# Autodesk Inventor assembly: WinchNM
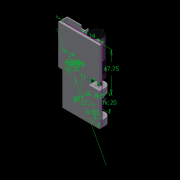
[picture p0: Inventor's stored thumbnail of the model, 180x180]
Saved by Autodesk Inventor 2019 (Build 230136000, 136)
## iProperties
Created: 2019-04-19
Part Number: WinchNM
Document SubType Name: Assembly
Designer: skylercleland
Author: skylercleland
## Documents named in this file (10)
- I:\FILES\School\12\DE\Projects\FinalProject\CAD\ShoeWinch\WinchNM.iam
- I:\FILES\School\12\DE\Projects\FinalProject\CAD\ShoeWinch\Bearing(8mm).ipt
- I:\FILES\School\12\DE\Projects\FinalProject\CAD\ShoeWinch\Bearing(608).ipt
- I:\FILES\School\12\DE\Projects\FinalProject\CAD\ShoeWinch\Part3.ipt
- I:\FILES\School\12\DE\Projects\FinalProject\CAD\ShoeWinch\Winch\Design Accelerator\Shaft2.iam
- I:\FILES\School\12\DE\Projects\FinalProject\CAD\ShoeWinch\Winch\Design Accelerator\Worm Gears2.iam
- I:\FILES\School\12\DE\Projects\FinalProject\CAD\ShoeWinch\Winch\Design Accelerator\Spur Gears2.iam
- I:\FILES\School\12\DE\Projects\FinalProject\CAD\ShoeWinch\LimitSwitch.ipt
- I:\FILES\School\12\DE\Projects\FinalProject\CAD\ShoeWinch\Part2NM.ipt
- I:\FILES\School\12\DE\Projects\FinalProject\CAD\ShoeWinch\MotorNM.ipt
## Components (10 placed, 9 different names)
1. Bearing(8mm):1 — Mate:20, Flush:7, Angle:4
2. Bearing(8mm):2 — Mate:21, Flush:8
3. Bearing(608):1 — Mate:6, Mate:7, Mate:17, Mate:18
4. Part3:1 — Mate:6, Mate:7, Mate:13, Tangent:1
5. Shaft:1 [sub-assembly] — Mate:15, Flush:4, Mate:22, Mate:23, Mate:24
6. Worm Gears:1 [sub-assembly] — Mate:13, Mate:19, Angle:4, Mate:22, Mate:23, Mate:24
7. Spur Gears:1 [sub-assembly] — Mate:15, Flush:4, Mate:28, Flush:10
8. LimitSwitch:1 — Tangent:1, Flush:9
9. Part2NM:1 — Mate:17, Mate:18, Mate:19, Mate:20, Flush:7, Mate:21, Flush:8, Flush:9, Mate:25, Mate:26, Mate:27
10. MotorNM:1 — Mate:25, Mate:26, Mate:27, Mate:28, Flush:10
## Relationships (23: Mate 16, Flush 5, Tangent 1, Angle 1)
- Mate:6: Bearing(608):1 ↔ Part3:1
- Mate:7: Bearing(608):1 ↔ Part3:1
- Mate:13: Part3:1 ↔ Worm Gears:1
- Mate:15: Shaft:1 ↔ Spur Gears:1
- Flush:4: Shaft:1 ↔ Spur Gears:1
- Tangent:1 (-1 mm): Part3:1 ↔ LimitSwitch:1
- Mate:17: Bearing(608):1 ↔ Part2NM:1
- Mate:18: Bearing(608):1 ↔ Part2NM:1
- Mate:19: Worm Gears:1 ↔ Part2NM:1
- Mate:20: Bearing(8mm):1 ↔ Part2NM:1
- Flush:7: Bearing(8mm):1 ↔ Part2NM:1
- Mate:21: Bearing(8mm):2 ↔ Part2NM:1
- Flush:8: Bearing(8mm):2 ↔ Part2NM:1
- Angle:4 (0 deg): Bearing(8mm):1 ↔ Worm Gears:1
- Mate:22: Shaft:1 ↔ Worm Gears:1
- Mate:23: Shaft:1 ↔ Worm Gears:1
- Mate:24: Shaft:1 ↔ Worm Gears:1
- Flush:9: LimitSwitch:1 ↔ Part2NM:1
- Mate:25: Part2NM:1 ↔ MotorNM:1
- Mate:26: Part2NM:1 ↔ MotorNM:1
- Mate:27: Part2NM:1 ↔ MotorNM:1
- Mate:28: Spur Gears:1 ↔ MotorNM:1
- Flush:10: Spur Gears:1 ↔ MotorNM:1
